# Autodesk Inventor assembly: kolo_napedowe
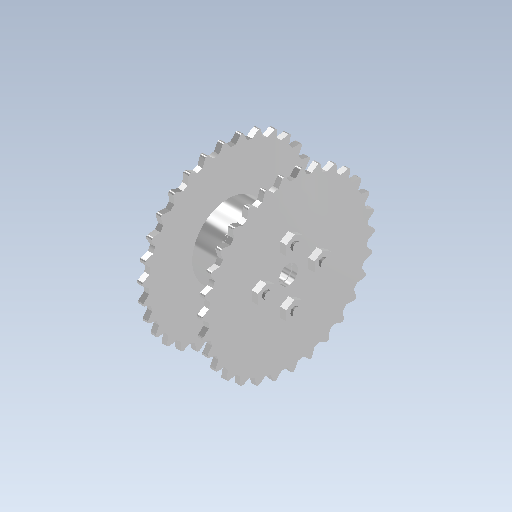
[picture p0: Inventor's stored thumbnail of the model, 512x512]
Saved by Autodesk Inventor 2020.3 (Build 243373000, 373)
## iProperties
Created: 2021-04-05
Part Number: kolo_napedowe
Document SubType Name: Assembly
Designer: patry
Mass: 134.226 g
Surface Area: 319.156 cm^2
Volume: 49.7132 cm^3
Density: 2.7 g/cm^3
Author: patry
## Documents named in this file (6)
- C:\Users\patry\Desktop\Konar staff\Ariadna2.1\ariadna_mechanika\Obszar roboczy\Naped\Kola\kolo_napedowe.iam
- C:\Users\patry\Desktop\Konar staff\Ariadna2.1\ariadna_mechanika\Obszar roboczy\Naped\Kola\kolo_zebate_duze_fi8.ipt
- C:\Users\patry\Desktop\Konar staff\Ariadna2.1\ariadna_mechanika\Obszar roboczy\Naped\Kola\piasta_kola_napedowego_fi8.ipt
- C:\Users\patry\Desktop\Konar staff\Ariadna2.1\ariadna_mechanika\Obszar roboczy\Naped\Sruby\M4_nut_3mm.ipt
- C:\Users\patry\Desktop\Konar staff\Ariadna2.1\ariadna_mechanika\Obszar roboczy\Naped\Sruby\M4x35.ipt
- C:\Users\patry\Desktop\Konar staff\Ariadna2.1\ariadna_mechanika\Obszar roboczy\Naped\Sruby\M5x15_docisk.ipt
## Components (13 placed, 5 different names)
1. kolo_zebate_duze_fi8:1 — Zestawiające:1, Zestawiające:2, Zestawiające:3, Zestawiające:8, Zestawiające:9, Zestawiające:13, Zestawiające:14, Zestawiające:15, Zestawiające:16, Zestawiające:17, Zestawiające:18
2. piasta_kola_napedowego_fi8:1 — Zestawiające:1, Zestawiające:2, Zestawiające:3, Zestawiające:4, Zestawiające:5, Zestawiające:6, Zestawiające:19, Styczny:1, Zestawiające:20, Styczny:2
3. kolo_zebate_duze_fi8:2 — Zestawiające:4, Zestawiające:5, Zestawiające:6
4. M4_nut_3mm:1 — Zestawiające:7, Równoległe:1
5. M4x35:1 — Zestawiające:7, Równoległe:1, Zestawiające:8, Zestawiające:9
6. M4_nut_3mm:2
7. M4x35:2 — Zestawiające:14, Zestawiające:18
8. M4_nut_3mm:3
9. M4x35:3 — Zestawiające:15, Zestawiające:16
10. M4_nut_3mm:4
11. M4x35:4 — Zestawiające:13, Zestawiające:17
12. M5x15_docisk:1 — Zestawiające:20, Styczny:2
13. M5x15_docisk:2 — Zestawiające:19, Styczny:1
## Relationships (26: Mate 20, Flush 4, Tangent 2)
- Zestawiające:1 [Mate]: kolo_zebate_duze_fi8:1 ↔ piasta_kola_napedowego_fi8:1
- Zestawiające:2 [Mate]: kolo_zebate_duze_fi8:1 ↔ piasta_kola_napedowego_fi8:1
- Zestawiające:3 [Mate]: kolo_zebate_duze_fi8:1 ↔ piasta_kola_napedowego_fi8:1
- Zestawiające:4 [Mate]: piasta_kola_napedowego_fi8:1 ↔ kolo_zebate_duze_fi8:2
- Zestawiające:5 [Mate]: piasta_kola_napedowego_fi8:1 ↔ kolo_zebate_duze_fi8:2
- Zestawiające:6 [Mate]: piasta_kola_napedowego_fi8:1 ↔ kolo_zebate_duze_fi8:2
- Zestawiające:7 [Mate]: M4_nut_3mm:1 ↔ M4x35:1
- Równoległe:1 [Flush] (1 mm): M4_nut_3mm:1 ↔ M4x35:1
- Zestawiające:8 [Mate]: kolo_zebate_duze_fi8:1 ↔ M4x35:1
- Zestawiające:9 [Mate]: kolo_zebate_duze_fi8:1 ↔ M4x35:1
- [Mate]: M4_nut_3mm:2 ↔ M4x35:2
- [Flush] (1 mm): M4_nut_3mm:2 ↔ M4x35:2
- [Mate]: M4_nut_3mm:3 ↔ M4x35:3
- [Flush] (1 mm): M4_nut_3mm:3 ↔ M4x35:3
- [Mate]: M4_nut_3mm:4 ↔ M4x35:4
- [Flush] (1 mm): M4_nut_3mm:4 ↔ M4x35:4
- Zestawiające:13 [Mate]: kolo_zebate_duze_fi8:1 ↔ M4x35:4
- Zestawiające:14 [Mate]: kolo_zebate_duze_fi8:1 ↔ M4x35:2
- Zestawiające:15 [Mate]: kolo_zebate_duze_fi8:1 ↔ M4x35:3
- Zestawiające:16 [Mate]: kolo_zebate_duze_fi8:1 ↔ M4x35:3
- Zestawiające:17 [Mate]: kolo_zebate_duze_fi8:1 ↔ M4x35:4
- Zestawiające:18 [Mate]: kolo_zebate_duze_fi8:1 ↔ M4x35:2
- Zestawiające:19 [Mate]: piasta_kola_napedowego_fi8:1 ↔ M5x15_docisk:2
- Styczny:1 [Tangent]: piasta_kola_napedowego_fi8:1 ↔ M5x15_docisk:2
- Zestawiające:20 [Mate]: piasta_kola_napedowego_fi8:1 ↔ M5x15_docisk:1
- Styczny:2 [Tangent]: piasta_kola_napedowego_fi8:1 ↔ M5x15_docisk:1
## Named parameters: d10_d6 = 0 mm, d11_d7 = 1 mm, d12_d6 = 0 mm, d13_d7 = 1 mm, d14_d6 = 0 mm, d15_d7 = 1 mm
